# Autodesk Inventor assembly: wheel with sprocket
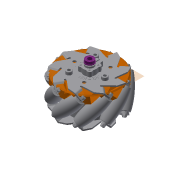
[picture p0: Inventor's stored thumbnail of the model, 180x180]
Saved by Autodesk Inventor 2018 (Build 220112000, 112)
## iProperties
Created: 2019-09-29
Part Number: wheel with sprocket
Document SubType Name: Assembly
Designer: ball
Author: ball
## Documents named in this file (5)
- C:\FTC\FTC8863CAD\2019 Robot\Mecanum Drive Train\wheel with sprocket.iam
- C:\FTC\FTC8863CAD\2019 Robot\Mecanum Drive Train\left wheel with clamping hub.iam
- C:\FTC\FTC8863CAD\Actobotics\615 parts\615102.ipt
- C:\FTC\FTC8863CAD\Actobotics\535 parts\535198.ipt
- C:\FTC\FTC8863CAD\Actobotics\633 parts\633104.ipt
## Components (6 placed, 4 different names)
1. left wheel with clamping hub:1 [sub-assembly] — Mate:1, Mate:2, Mate:3, Mate:4, Mate:5, Mate:9, Mate:10, Mate:11
2. 615102:1 — Mate:1, Mate:2, Mate:3, Mate:7, Mate:13, Mate:14
3. 535198:1 — Mate:9, Mate:12
4. 535198:2 — Mate:7, Mate:15
5. 633104:1 — Mate:10, Mate:11, Mate:12
6. 633104:2 — Mate:13, Mate:14, Mate:15
## Relationships (13: Mate 13)
- Mate:1: left wheel with clamping hub:1 ↔ 615102:1
- Mate:2: left wheel with clamping hub:1 ↔ 615102:1
- Mate:3 (2.54 mm): left wheel with clamping hub:1 ↔ 615102:1
- Mate:4: left wheel with clamping hub:1
- Mate:5: left wheel with clamping hub:1
- Mate:7: 615102:1 ↔ 535198:2
- Mate:9: left wheel with clamping hub:1 ↔ 535198:1
- Mate:10: left wheel with clamping hub:1 ↔ 633104:1
- Mate:11: left wheel with clamping hub:1 ↔ 633104:1
- Mate:12: 535198:1 ↔ 633104:1
- Mate:13: 615102:1 ↔ 633104:2
- Mate:14: 615102:1 ↔ 633104:2
- Mate:15: 535198:2 ↔ 633104:2
